# Autodesk Inventor assembly: Controller_Unit
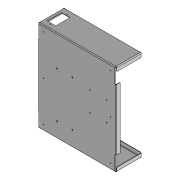
[picture p0: Inventor's stored thumbnail of the model, 180x180]
Saved by Autodesk Inventor 2020 (Build 240168000, 168)
## iProperties
Created: 2021-08-23
Part Number: Controller_Unit
Document SubType Name: Assembly
Designer: magnarecta
Author: magnarecta
## Documents named in this file (4)
- C:\Users\lvglv\Documents\GitHub\Vibration_Generator\Asem\Controller_Unit.iam
- C:\Users\lvglv\Documents\GitHub\Vibration_Generator\Parts\Meviy\Controller_A.ipt
- C:\Users\lvglv\Documents\GitHub\Vibration_Generator\Parts\Oriental_motor\A1806\A1806.ipt
- C:\Users\lvglv\Documents\GitHub\Vibration_Generator\Parts\Meviy\ridgidbot-big-power-suppply-upgrade-1.snapshot.3\SE-450-24.ipt
## Components (3 placed, 3 different names)
1. Controller_A:1 — 挿入:1, 挿入:2, 挿入:3, メイト:1
2. A1806:1 — 挿入:3, メイト:1
3. SE-450-24:1 — 挿入:1, 挿入:2
## Relationships (4: Insert 3, Mate 1)
- 挿入:1 [Insert]: Controller_A:1 ↔ SE-450-24:1
- 挿入:2 [Insert]: Controller_A:1 ↔ SE-450-24:1
- 挿入:3 [Insert]: Controller_A:1 ↔ A1806:1
- メイト:1 [Mate]: Controller_A:1 ↔ A1806:1
